# Autodesk Inventor assembly: small pulley assembly
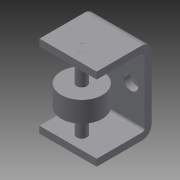
[picture p0: Inventor's stored thumbnail of the model, 180x180]
Saved by Autodesk Inventor 2013 (Build 170138000, 138)
## iProperties
Created: 2013-02-01
Part Number: small pulley assembly
Document SubType Name: Assembly
Designer: Arpan
Author: Arpan
## Documents named in this file (4)
- C:\Users\Arpan\Documents\GitHub\frc2013CAD\Cimber actual\small pulley assembly.iam
- C:\Users\Arpan\Documents\GitHub\frc2013CAD\Cimber actual\pulley mount. actual ipt.ipt
- C:\Users\Arpan\Documents\GitHub\frc2013CAD\Cimber actual\3 16ths shaft.ipt
- C:\Users\Arpan\Documents\GitHub\frc2013CAD\Cimber actual\1 8th pulley.ipt
## Components (3 placed, 3 different names)
1. pulley mount. actual ipt:1 — Mate:1, Flush:1
2. 3 16ths shaft:1 — Mate:1, Flush:1, Mate:2
3. 1 8th pulley:1 — Mate:2
## Relationships (3: Mate 2, Flush 1)
- Mate:1: pulley mount. actual ipt:1 ↔ 3 16ths shaft:1
- Flush:1: pulley mount. actual ipt:1 ↔ 3 16ths shaft:1
- Mate:2: 3 16ths shaft:1 ↔ 1 8th pulley:1
